# Autodesk Inventor assembly: RT_FRM_A_003_FrameV4
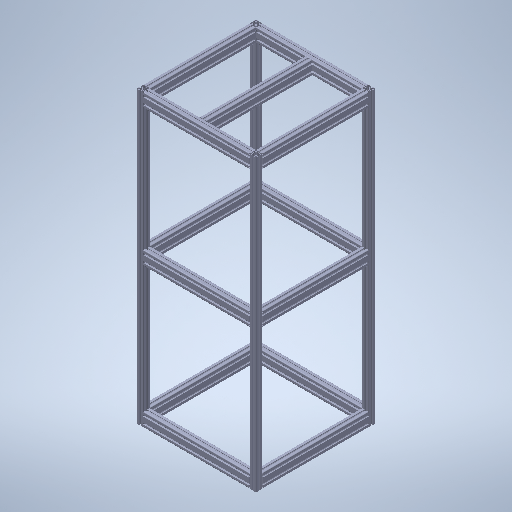
[picture p0: Inventor's stored thumbnail of the model, 512x512]
Saved by Autodesk Inventor 2025.4 (Build 294407000, 407)
## iProperties
Created: 2026-07-11
Part Number: RT_FRM_A_003_FrameV4
Document SubType Name: Assembly
Designer: louis
Author: louis
## Documents named in this file (3)
- C:\Users\louis\OneDrive\Desktop\R_Trident\02_CAD\04_Subassemblies\RT_FRM_A_003_FrameV4.iam
- C:\Users\louis\OneDrive\Desktop\R_Trident\02_CAD\01_Standard_Parts\02_FRM_Extrusions_Frame_V4\4040x1600.ipt
- C:\Users\louis\OneDrive\Desktop\R_Trident\02_CAD\01_Standard_Parts\02_FRM_Extrusions_Frame_V4\4080x500.ipt
## Components (17 placed, 2 different names)
1. 4040x1600:1 — Flush:2, Flush:3, Flush:14, Flush:15, Mate:3, Mate:4, Mate:9, Flush:17, Flush:24, Flush:25, Flush:26, Flush:31, Mate:18
2. 4040x1600:2 — Flush:4, Flush:5, Flush:12, Flush:16, Mate:6, Flush:18, Flush:20, Flush:27, Mate:14, Mate:15, Flush:30, Mate:17, Flush:33, Mate:20
3. 4040x1600:3 — Flush:1, Flush:8, Mate:1, Flush:9, Flush:13, Mate:5, Mate:7, Flush:22, Flush:23, Mate:13, Mate:16, Flush:32, Mate:19
4. 4040x1600:4 — Flush:6, Flush:7, Mate:2, Flush:10, Flush:11, Mate:8, Flush:19, Flush:21, Flush:28
5. 4080x500:1 — Flush:1, Flush:2, Flush:13, Flush:14, Mate:3, Mate:5, Symmetry:1
6. 4080x500:2 — Flush:3, Flush:4, Flush:15, Flush:16, Mate:4, Symmetry:2
7. 4080x500:3 — Flush:5, Flush:6, Flush:11, Flush:12, Mate:6, Symmetry:1
8. 4080x500:4 — Flush:7, Flush:8, Mate:1, Mate:2, Flush:9, Flush:10, Symmetry:2, Mate:25, Flush:34
9. 4080x500:5 — Flush:17, Flush:18, Flush:26, Mate:15
10. 4080x500:6 — Flush:23, Flush:24, Flush:25, Mate:16
11. 4080x500:7 — Flush:21, Flush:22, Flush:28, Mate:13
12. 4080x500:8 — Flush:19, Flush:20, Flush:27, Mate:14
13. 4080x500:9 — Flush:30, Mate:17, Mate:23
14. 4080x500:10 — Flush:31, Mate:18, Mate:24
15. 4080x500:11 — Flush:32, Mate:19, Mate:22
16. 4080x500:12 — Flush:33, Mate:20, Mate:21
17. 4080x500:13 — Mate:25, Flush:34, Mate:26
## Relationships (62: Flush 34, Mate 26, Symmetry 2)
- Flush:1: 4040x1600:3 ↔ 4080x500:1
- Flush:2: 4040x1600:1 ↔ 4080x500:1
- Flush:3: 4040x1600:1 ↔ 4080x500:2
- Flush:4: 4040x1600:2 ↔ 4080x500:2
- Flush:5: 4040x1600:2 ↔ 4080x500:3
- Flush:6: 4040x1600:4 ↔ 4080x500:3
- Flush:7: 4040x1600:4 ↔ 4080x500:4
- Flush:8: 4040x1600:3 ↔ 4080x500:4
- Mate:1: 4040x1600:3 ↔ 4080x500:4
- Mate:2: 4040x1600:4 ↔ 4080x500:4
- Flush:9: 4040x1600:3 ↔ 4080x500:4
- Flush:10: 4040x1600:4 ↔ 4080x500:4
- Flush:11: 4040x1600:4 ↔ 4080x500:3
- Flush:12: 4040x1600:2 ↔ 4080x500:3
- Flush:13: 4040x1600:3 ↔ 4080x500:1
- Flush:14: 4040x1600:1 ↔ 4080x500:1
- Flush:15: 4040x1600:1 ↔ 4080x500:2
- Flush:16: 4040x1600:2 ↔ 4080x500:2
- Mate:3: 4040x1600:1 ↔ 4080x500:1
- Mate:4: 4040x1600:1 ↔ 4080x500:2
- Mate:5: 4040x1600:3 ↔ 4080x500:1
- Mate:6: 4040x1600:2 ↔ 4080x500:3
- Symmetry:1: 4080x500:1 ↔ 4080x500:3
- Symmetry:2: 4080x500:2 ↔ 4080x500:4
- Mate:7: 4040x1600:3
- Mate:8: 4040x1600:4
- Mate:9: 4040x1600:1
- Mate:10
- Mate:11
- Mate:12
- Flush:17: 4040x1600:1 ↔ 4080x500:5
- Flush:18: 4040x1600:2 ↔ 4080x500:5
- Flush:19: 4040x1600:4 ↔ 4080x500:8
- Flush:20: 4040x1600:2 ↔ 4080x500:8
- Flush:21: 4040x1600:4 ↔ 4080x500:7
- Flush:22: 4040x1600:3 ↔ 4080x500:7
- Flush:23: 4040x1600:3 ↔ 4080x500:6
- Flush:24: 4040x1600:1 ↔ 4080x500:6
- Flush:25: 4040x1600:1 ↔ 4080x500:6
- Flush:26: 4040x1600:1 ↔ 4080x500:5
- Flush:27: 4040x1600:2 ↔ 4080x500:8
- Flush:28: 4040x1600:4 ↔ 4080x500:7
- Mate:13: 4040x1600:3 ↔ 4080x500:7
- Mate:14: 4040x1600:2 ↔ 4080x500:8
- Mate:15: 4040x1600:2 ↔ 4080x500:5
- Mate:16: 4040x1600:3 ↔ 4080x500:6
- Flush:29 (800 mm)
- Flush:30: 4040x1600:2 ↔ 4080x500:9
- Mate:17: 4040x1600:2 ↔ 4080x500:9
- Flush:31: 4040x1600:1 ↔ 4080x500:10
- Mate:18: 4040x1600:1 ↔ 4080x500:10
- Flush:32: 4040x1600:3 ↔ 4080x500:11
- Mate:19: 4040x1600:3 ↔ 4080x500:11
- Flush:33: 4040x1600:2 ↔ 4080x500:12
- Mate:20: 4040x1600:2 ↔ 4080x500:12
- Mate:21: 4080x500:12
- Mate:22: 4080x500:11
- Mate:23: 4080x500:9
- Mate:24: 4080x500:10
- Mate:25: 4080x500:4 ↔ 4080x500:13
- Flush:34: 4080x500:4 ↔ 4080x500:13
- Mate:26: 4080x500:13
